# Autodesk Inventor assembly: 000 ASY GBK Gubkinskiy
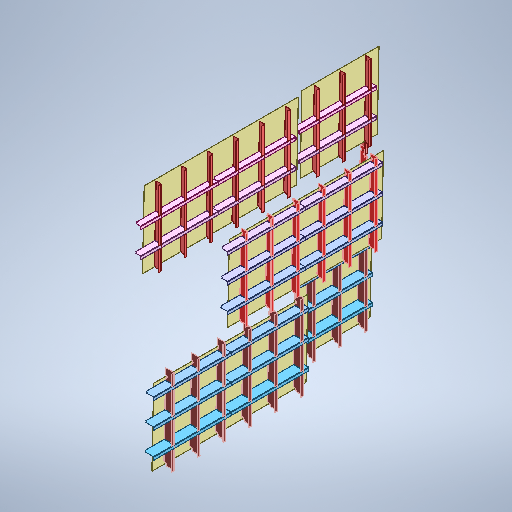
[picture p0: Inventor's stored thumbnail of the model, 512x512]
Saved by Autodesk Inventor 2026 (Build 300175000, 175)
## iProperties
Created: 2026-04-17
Part Number: 000 ASY GBK Gubkinskiy
Document SubType Name: Assembly
Designer: admin
Author: admin
## Documents named in this file (12)
- C:\Users\pokla\Documents\Inventor\GBK-Gubkinskiy\000 ASY GBK Gubkinskiy.iam
- C:\Users\pokla\Documents\Inventor\GBK-Gubkinskiy\GBK bottom.ipt
- C:\Users\pokla\Documents\Inventor\GBK-Gubkinskiy\01 ASY GBK wall shield 1.1.1.iam
- C:\Users\pokla\Documents\Inventor\GBK-Gubkinskiy\GBK dummy wall 1.ipt
- C:\Users\pokla\Documents\Inventor\GBK-Gubkinskiy\GBK dummy wall 4.ipt
- C:\Users\pokla\Documents\Inventor\GBK-Gubkinskiy\GBK overall model.ipt
- C:\Users\pokla\Documents\Inventor\GBK-Gubkinskiy\02.1 GBK main rib.ipt
- C:\Users\pokla\Documents\Inventor\GBK-Gubkinskiy\03.1 GBK main3  rib.ipt
- C:\Users\pokla\Documents\Inventor\GBK-Gubkinskiy\02 ASY GBK wall shield 1.1.2.iam
- C:\Users\pokla\Documents\Inventor\GBK-Gubkinskiy\04 ASY GBK wall shield 1.2.4.iam
- C:\Users\pokla\Documents\Inventor\GBK-Gubkinskiy\07 ASY GBK wall shield 1.3.1.iam
- C:\Users\pokla\Documents\Inventor\GBK-Gubkinskiy\08 ASY GBK wall shield 1.3.8.iam
## Components (12 placed, 11 different names)
1. GBK bottom.ipt:1 — Совмещение:10, Совмещение:11, Совмещение:12, Совмещение:13, Совмещение:14, Жесткий:1
2. 01 ASY GBK wall shield 1.1.1.iam:1 [sub-assembly]
3. GBK dummy wall 1.ipt:1 — Совмещение:10
4. GBK dummy wall 1.ipt:2 — Совмещение:11, Совмещение:12
5. GBK dummy wall 4.ipt:1 — Совмещение:13, Совмещение:14
6. GBK overall model:1 — Жесткий:1
7. 02.1 GBK main rib:1 — Жесткий:3
8. 03.1 GBK main3  rib:1 — Жесткий:3
9. 02 ASY GBK wall shield 1.1.2:1 [sub-assembly]
10. 04 ASY GBK wall shield 1.2.4:1 [sub-assembly]
11. 07 ASY GBK wall shield 1.3.1:1 [sub-assembly]
12. 08 ASY GBK wall shield 1.3.8:1 [sub-assembly]
## Relationships (11: Mate 6, Flush 2, WeldJoint 2, RevoluteJoint 1)
- [Flush]: GBK bottom.ipt:1 ↔ 01 ASY GBK wall shield 1.1.1.iam:1
- [Mate]: GBK bottom.ipt:1 ↔ 01 ASY GBK wall shield 1.1.1.iam:1
- Совмещение:10 [Mate]: GBK bottom.ipt:1 ↔ GBK dummy wall 1.ipt:1
- Совмещение:11 [Mate]: GBK bottom.ipt:1 ↔ GBK dummy wall 1.ipt:2
- Совмещение:12 [Mate]: GBK bottom.ipt:1 ↔ GBK dummy wall 1.ipt:2
- Совмещение:13 [Mate]: GBK bottom.ipt:1 ↔ GBK dummy wall 4.ipt:1
- Совмещение:14 [Mate]: GBK bottom.ipt:1 ↔ GBK dummy wall 4.ipt:1
- Жесткий:1 [WeldJoint]: GBK bottom.ipt:1 ↔ GBK overall model:1
- [RevoluteJoint]: 01 ASY GBK wall shield 1.1.1.iam:1 ↔ 02.1 GBK main rib:1
- Жесткий:3 [WeldJoint]: 02.1 GBK main rib:1 ↔ 03.1 GBK main3  rib:1
- [Flush]: 01 ASY GBK wall shield 1.1.1.iam:1 ↔ 02.1 GBK main rib:1
